# Autodesk Inventor assembly: AK60-6
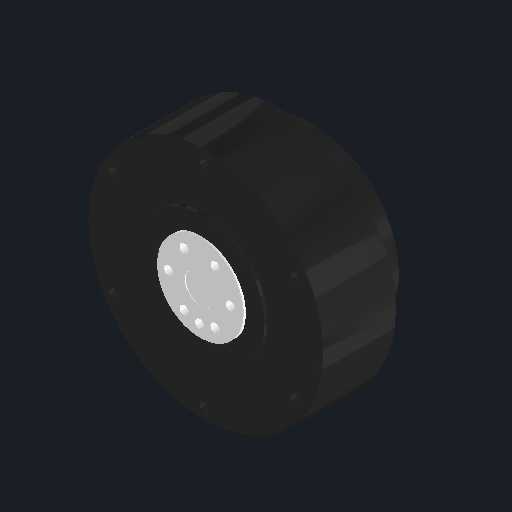
[picture p0: Inventor's stored thumbnail of the model, 512x512]
Saved by Autodesk Inventor 2023 (Build 270158000, 158)
## iProperties
Created: 2023-02-15
Part Number: AK60-6
Document SubType Name: Assembly
Designer: dzw04
Author: dzw04
## Documents named in this file (3)
- C:\Users\dzw04\Saxion\Mechatronica Lectoraat LMECH LED - Testomgeving van Dion\Component_Database\SAM2\01. Drawings\Components\AK60-6.iam
- C:\Users\dzw04\Saxion\Mechatronica Lectoraat LMECH LED - Testomgeving van Dion\Component_Database\SAM2\01. Drawings\Components\Stator.ipt
- C:\Users\dzw04\Saxion\Mechatronica Lectoraat LMECH LED - Testomgeving van Dion\Component_Database\SAM2\01. Drawings\Components\Rotor.ipt
## Components (2 placed, 2 different names)
1. Stator:1 — Rotational:1
2. Rotor:1 — Rotational:1
## Relationships (1: RevoluteJoint 1)
- Rotational:1 [RevoluteJoint] (0.5 mm): Stator:1 ↔ Rotor:1
